# Autodesk Inventor assembly: Structure
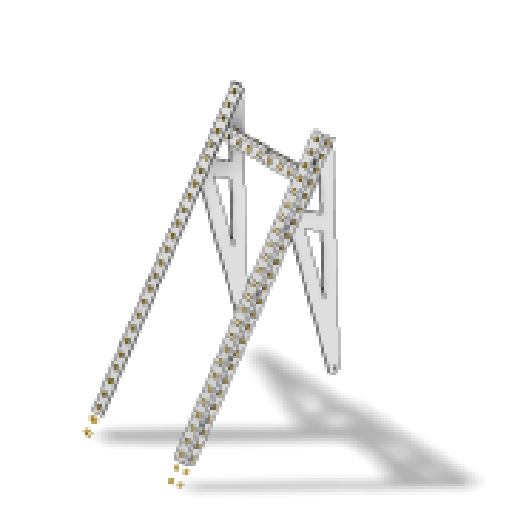
[picture p0: Inventor's stored thumbnail of the model, 512x512]
Saved by Autodesk Inventor 2025.2 (Build 292293000, 293)
## iProperties
Created: 2025-02-15
Part Number: Structure
Document SubType Name: Assembly
Designer: Averey Ku
Author: Averey Ku
## Documents named in this file (5)
- C:\Users\avere\VEX-CAD\V5-CAD\Conveyer\Structure.iam
- C:\Users\avere\VEX-CAD\V5-CAD\Conveyer\Custom Parts\Triangle Gusset.ipt
- C:\Users\avere\VEX-CAD\ROBOPROS-CAD-Inventor\Motion\Shaft LS\Bearing Flat Low Profile.ipt
- C:\Users\avere\VEX-CAD\ROBOPROS-CAD-Inventor\Structure\Angle\Aluminum 1x1\Alu Angle 1x1x9.ipt
- C:\Users\avere\VEX-CAD\ROBOPROS-CAD-Inventor\Structure\C Channel\Aluminum 1x3x1 Half\Alu C Half 1x3x1x27.ipt
## Components (7 placed, 4 different names)
1. Triangle Gusset:1
2. Triangle Gusset:2
3. Bearing Flat Low Profile:1 — Insert:2, Mate:10
4. Bearing Flat Low Profile:2 — Insert:1, Mate:9
5. Alu Angle 1x1x9:1
6. Alu C Half 1x3x1x27:1 — Insert:1, Mate:9
7. Alu C Half 1x3x1x27:2 — Insert:2, Mate:10
## Relationships (4: Insert 2, Mate 2)
- Insert:1 (1.5875 mm): Bearing Flat Low Profile:2 ↔ Alu C Half 1x3x1x27:1
- Mate:9: Bearing Flat Low Profile:2 ↔ Alu C Half 1x3x1x27:1
- Insert:2 (1.5875 mm): Bearing Flat Low Profile:1 ↔ Alu C Half 1x3x1x27:2
- Mate:10: Bearing Flat Low Profile:1 ↔ Alu C Half 1x3x1x27:2
